# Autodesk Inventor assembly: !wing_MIR
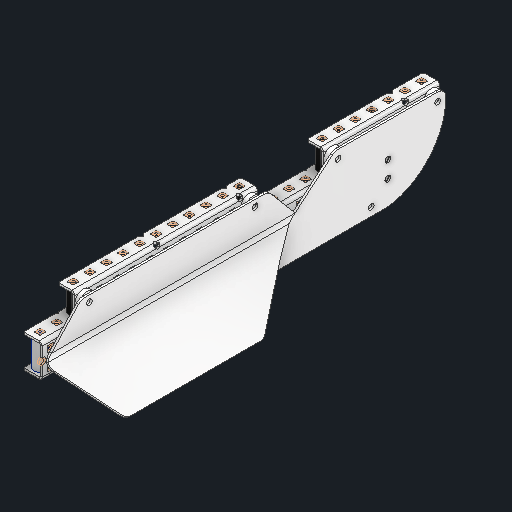
[picture p0: Inventor's stored thumbnail of the model, 512x512]
Saved by Autodesk Inventor 2024 (Build 280153000, 153)
## iProperties
Created: 2023-10-18
Part Number: !wing_MIR
Document SubType Name: Assembly
Designer: Averey Ku
Author: Averey Ku
## Documents named in this file (17)
- D:\vex_robotics\hardware\cad\goated_v0.1\chassis\mirrored_parts\!wing_MIR.iam
- D:\vex_robotics\hardware\cad\goated_v0.1\chassis\mirrored_parts\Alu C 1x2x1x22_MIR.ipt
- D:\vex_robotics\hardware\cad\goated_v0.1\chassis\mirrored_parts\Alu Angle 1x1x7_MIR.ipt
- D:\vex_robotics\hardware\cad\VEX-CAD-Inventor-1.41\Structure\Standoff\Standoff .75.ipt
- D:\vex_robotics\hardware\cad\VEX-CAD-Inventor-1.41\Structure\Standoff.ipt
- D:\vex_robotics\hardware\cad\goated_v0.1\chassis\mirrored_parts\sled_MIR.ipt
- D:\vex_robotics\hardware\cad\VEX-CAD-Inventor-1.41\Motion\Spacers\Spacer Nylon .375 OD\NSpacer .375 OD x .375.ipt
- D:\vex_robotics\hardware\cad\VEX-CAD-Inventor-1.41\Motion\Spacers\Spacer Nylon .375 OD.ipt
- D:\vex_robotics\hardware\cad\VEX-CAD-Inventor-1.41\Motion\Spacers\Washer Teflon\TWasher .375 OD x .04000.ipt
- D:\vex_robotics\hardware\cad\VEX-CAD-Inventor-1.41\Motion\Spacers\Washer Teflon.ipt
- D:\vex_robotics\hardware\cad\VEX-CAD-Inventor-1.41\Motion\Spacers\Washer Steel\SWasher .375 OD x .015625.ipt
- D:\vex_robotics\hardware\cad\VEX-CAD-Inventor-1.41\Motion\Spacers\Washer Steel.ipt
- D:\vex_robotics\hardware\cad\goated_v0.1\chassis\mirrored_parts\.375 OD Aluminum Spacer 0.875_MIR.ipt
- D:\vex_robotics\hardware\cad\VEX-CAD-Inventor-1.41\Motion\Spacers\Spacer Nylon .500 OD\NSpacer White .500 OD x .125.ipt
- D:\vex_robotics\hardware\cad\VEX-CAD-Inventor-1.41\Motion\Spacers\Spacer Nylon .500 OD.ipt
- D:\vex_robotics\hardware\cad\goated_v0.1\chassis\mirrored_parts\Alu Angle 1x1x11_MIR.ipt
- D:\vex_robotics\hardware\cad\goated_v0.1\chassis\mirrored_parts\wedge_MIR.ipt
## Components (29 placed, 11 different names)
1. Alu C 1x2x1x22_MIR:1 — Insert:1, Insert:2, Insert:12, Insert:13, Insert:14, Insert:16, Insert:17, Mate:4, Insert:20, Insert:24, Insert:25, Insert:26, Insert:27, Insert:28
2. Alu Angle 1x1x7_MIR:1 — Insert:3, Mate:1, Mate:2, Insert:4, Insert:15
3. Standoff .75:1 — Insert:3, Insert:1
4. Standoff .75:2 — Mate:1, Insert:2
5. sled_MIR:1 — Mate:2, Insert:4, Mate:3, Insert:5, Insert:18, Insert:19
6. Alu Angle 1x1x7_MIR:2 — Mate:3, Insert:5
7. NSpacer .375 OD x .375:1 — Insert:12, Insert:8
8. TWasher .375 OD x .04000:1 — Insert:7, Insert:6
9. TWasher .375 OD x .04000:2 — Insert:8, Insert:7
10. SWasher .375 OD x .015625:1 — Insert:6
11. NSpacer .375 OD x .375:2 — Insert:13, Insert:11
12. TWasher .375 OD x .04000:3 — Insert:10, Insert:9
13. TWasher .375 OD x .04000:4 — Insert:11, Insert:10
14. SWasher .375 OD x .015625:2 — Insert:9
15. .375 OD Aluminum Spacer 0.875_MIR:1 — Insert:14
16. NSpacer White .500 OD x .125:1 — Insert:16
17. NSpacer White .500 OD x .125:2 — Insert:18
18. NSpacer White .500 OD x .125:3 — Insert:17
19. NSpacer White .500 OD x .125:4 — Insert:15
20. NSpacer White .500 OD x .125:5 — Insert:19
21. Alu Angle 1x1x11_MIR:1 — Mate:4, Insert:20, Mate:5, Insert:21
22. wedge_MIR:1 — Mate:5, Insert:21, Insert:22, Insert:23
23. NSpacer White .500 OD x .125:6 — Insert:22
24. NSpacer White .500 OD x .125:7 — Insert:23
25. Standoff .75:3 — Insert:24
26. Standoff .75:4 — Insert:25
27. .375 OD Aluminum Spacer 0.875_MIR:2 — Insert:26
28. .375 OD Aluminum Spacer 0.875_MIR:3 — Insert:27
29. .375 OD Aluminum Spacer 0.875_MIR:4 — Insert:28
## Relationships (33: Insert 28, Mate 5)
- Insert:3: Alu Angle 1x1x7_MIR:1 ↔ Standoff .75:1
- Insert:1: Alu C 1x2x1x22_MIR:1 ↔ Standoff .75:1
- Mate:1: Alu Angle 1x1x7_MIR:1 ↔ Standoff .75:2
- Insert:2: Alu C 1x2x1x22_MIR:1 ↔ Standoff .75:2
- Mate:2: Alu Angle 1x1x7_MIR:1 ↔ sled_MIR:1
- Insert:4 (3.175 mm): Alu Angle 1x1x7_MIR:1 ↔ sled_MIR:1
- Mate:3: sled_MIR:1 ↔ Alu Angle 1x1x7_MIR:2
- Insert:5 (3.175 mm): sled_MIR:1 ↔ Alu Angle 1x1x7_MIR:2
- Insert:12: Alu C 1x2x1x22_MIR:1 ↔ NSpacer .375 OD x .375:1
- Insert:8: NSpacer .375 OD x .375:1 ↔ TWasher .375 OD x .04000:2
- Insert:7: TWasher .375 OD x .04000:1 ↔ TWasher .375 OD x .04000:2
- Insert:6: TWasher .375 OD x .04000:1 ↔ SWasher .375 OD x .015625:1
- Insert:13: Alu C 1x2x1x22_MIR:1 ↔ NSpacer .375 OD x .375:2
- Insert:11: NSpacer .375 OD x .375:2 ↔ TWasher .375 OD x .04000:4
- Insert:10: TWasher .375 OD x .04000:3 ↔ TWasher .375 OD x .04000:4
- Insert:9: TWasher .375 OD x .04000:3 ↔ SWasher .375 OD x .015625:2
- Insert:14: Alu C 1x2x1x22_MIR:1 ↔ .375 OD Aluminum Spacer 0.875_MIR:1
- Insert:16: Alu C 1x2x1x22_MIR:1 ↔ NSpacer White .500 OD x .125:1
- Insert:18: sled_MIR:1 ↔ NSpacer White .500 OD x .125:2
- Insert:17: Alu C 1x2x1x22_MIR:1 ↔ NSpacer White .500 OD x .125:3
- Insert:15: Alu Angle 1x1x7_MIR:1 ↔ NSpacer White .500 OD x .125:4
- Insert:19: sled_MIR:1 ↔ NSpacer White .500 OD x .125:5
- Mate:4: Alu C 1x2x1x22_MIR:1 ↔ Alu Angle 1x1x11_MIR:1
- Insert:20 (19.05 mm): Alu C 1x2x1x22_MIR:1 ↔ Alu Angle 1x1x11_MIR:1
- Mate:5: Alu Angle 1x1x11_MIR:1 ↔ wedge_MIR:1
- Insert:21 (3.175 mm): Alu Angle 1x1x11_MIR:1 ↔ wedge_MIR:1
- Insert:22: wedge_MIR:1 ↔ NSpacer White .500 OD x .125:6
- Insert:23: wedge_MIR:1 ↔ NSpacer White .500 OD x .125:7
- Insert:24: Alu C 1x2x1x22_MIR:1 ↔ Standoff .75:3
- Insert:25: Alu C 1x2x1x22_MIR:1 ↔ Standoff .75:4
- Insert:26: Alu C 1x2x1x22_MIR:1 ↔ .375 OD Aluminum Spacer 0.875_MIR:2
- Insert:27: Alu C 1x2x1x22_MIR:1 ↔ .375 OD Aluminum Spacer 0.875_MIR:3
- Insert:28: Alu C 1x2x1x22_MIR:1 ↔ .375 OD Aluminum Spacer 0.875_MIR:4
